# Autodesk Inventor assembly: DC_Servo_JGB37-520
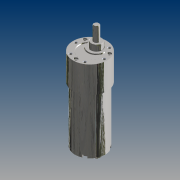
[picture p0: Inventor's stored thumbnail of the model, 180x180]
Saved by Autodesk Inventor 2021 (Build 250183000, 183)
## iProperties
Created: 2017-03-25
Part Number: DC_Servo_JGB37-520
Document SubType Name: Assembly
Designer: Admin
Mass: 100.69 g
Surface Area: 201.705 cm^2
Volume: 16.0056 cm^3
Density: 6.2909 g/cm^3
Sending System: SolidWorks 2017
Last Author: User
Last Saved: 2017-03-27
Author: Admin
## Documents named in this file (9)
- C:\Users\Admin\Desktop\DO_AN_TOT_NGHIEP_2024\Mechanical\Design_in_3D\Library\DC_Servo_JGB37-520.iam
- C:\Users\Admin\Downloads\jgb37-520-1.snapshot.2\GEARED BODY, MOTOR, JGB37-520.ipt
- C:\Users\Admin\Downloads\jgb37-520-1.snapshot.2\DC MOTOR, JGB37-520.ipt
- C:\Users\Admin\Downloads\jgb37-520-1.snapshot.2\MOTOR SHAFT, JGB37-520.ipt
- C:\Users\Admin\Downloads\jgb37-520-1.snapshot.2\SHAFT COUPLER, JGB37-520.ipt
- C:\Users\Admin\Downloads\jgb37-520-1.snapshot.2\COUPLING BRACKET, GEARED BODY TO DC MOTOR, JGB37-520.ipt
- C:\Users\Admin\Downloads\jgb37-520-1.snapshot.2\PLASTIC COVER, DC MOTOR, JGB37-520.ipt
- C:\Users\Admin\Downloads\jgb37-520-1.snapshot.2\CONNECTION, DC MOTOR, JGB37-520.ipt
- C:\Users\Admin\Downloads\jgb37-520-1.snapshot.2\PLASTIC COVER, DC MOTOR, JGB37-520_CPY.ipt
## Components (9 placed, 8 different names)
1. GEARED BODY, MOTOR, JGB37-520:1
2. DC MOTOR, JGB37-520:1 — Insert:1
3. MOTOR SHAFT, JGB37-520:1
4. SHAFT COUPLER, JGB37-520:1
5. COUPLING BRACKET, GEARED BODY TO DC MOTOR, JGB37-520:1
6. PLASTIC COVER, DC MOTOR, JGB37-520:1
7. CONNECTION, DC MOTOR, JGB37-520:1 — Mate:3, Flush:4, Mate:4
8. CONNECTION, DC MOTOR, JGB37-520:2 — Mate:1, Mate:2, Flush:1
9. PLASTIC COVER, DC MOTOR, JGB37-520_CPY:1 — Insert:1, Mate:1, Mate:2, Flush:1, Mate:3, Flush:4, Mate:4
## Relationships (7: Mate 4, Flush 2, Insert 1)
- Insert:1: DC MOTOR, JGB37-520:1 ↔ PLASTIC COVER, DC MOTOR, JGB37-520_CPY:1
- Mate:1: CONNECTION, DC MOTOR, JGB37-520:2 ↔ PLASTIC COVER, DC MOTOR, JGB37-520_CPY:1
- Mate:2: CONNECTION, DC MOTOR, JGB37-520:2 ↔ PLASTIC COVER, DC MOTOR, JGB37-520_CPY:1
- Flush:1: CONNECTION, DC MOTOR, JGB37-520:2 ↔ PLASTIC COVER, DC MOTOR, JGB37-520_CPY:1
- Mate:3: CONNECTION, DC MOTOR, JGB37-520:1 ↔ PLASTIC COVER, DC MOTOR, JGB37-520_CPY:1
- Flush:4: CONNECTION, DC MOTOR, JGB37-520:1 ↔ PLASTIC COVER, DC MOTOR, JGB37-520_CPY:1
- Mate:4: CONNECTION, DC MOTOR, JGB37-520:1 ↔ PLASTIC COVER, DC MOTOR, JGB37-520_CPY:1
